# Autodesk Inventor assembly: Magazine
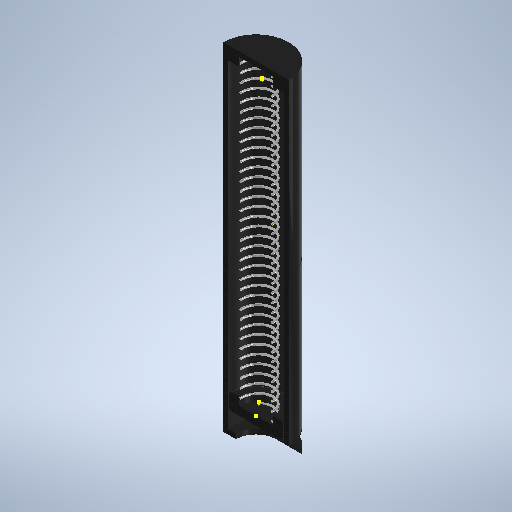
[picture p0: Inventor's stored thumbnail of the model, 512x512]
Saved by Autodesk Inventor 2025.1 (Build 291241020, 241B)
## iProperties
Created: 2024-11-13
Part Number: Magazine
Document SubType Name: Assembly
Designer: leon-
Mass: 105.142 g
Surface Area: 579.469 cm^2
Volume: 79.933 cm^3
Density: 1.31537 g/cm^3
Author: leon-
## Documents named in this file (5)
- C:\Users\leon-\OneDrive\Dokumente\Education\Berkeley\Embedded_Systems\Project\MagDrop4\CAD_Model\Magazine.iam
- C:\Users\leon-\OneDrive\Dokumente\Education\Berkeley\Embedded_Systems\Project\MagDrop4\CAD_Model\Purchase_Parts\Mechanical\Spring.ipt
- C:\Users\leon-\OneDrive\Dokumente\Education\Berkeley\Embedded_Systems\Project\MagDrop4\CAD_Model\3DPrint_Parts\Spring_Top.ipt
- C:\Users\leon-\OneDrive\Dokumente\Education\Berkeley\Embedded_Systems\Project\MagDrop4\CAD_Model\3DPrint_Parts\Magazine_Tube_1.ipt
- C:\Users\leon-\OneDrive\Dokumente\Education\Berkeley\Embedded_Systems\Project\MagDrop4\CAD_Model\3DPrint_Parts\Magazine_Tube_2.ipt
## Components (4 placed, 4 different names)
1. Spring:1 — Mate:3, Mate:4, Mate:6, Mate:9
2. Spring_Top:1 — Mate:3, Mate:4, Mate:5
3. Magazine_Tube_1:1 — Mate:5, Mate:6, Mate:7, Mate:8
4. Magazine_Tube_2:1 — Mate:7, Mate:8
## Relationships (7: Mate 7)
- Mate:3: Spring:1 ↔ Spring_Top:1
- Mate:4: Spring:1 ↔ Spring_Top:1
- Mate:5: Spring_Top:1 ↔ Magazine_Tube_1:1
- Mate:6: Spring:1 ↔ Magazine_Tube_1:1
- Mate:7: Magazine_Tube_1:1 ↔ Magazine_Tube_2:1
- Mate:8: Magazine_Tube_1:1 ↔ Magazine_Tube_2:1
- Mate:9: Spring:1
